# Autodesk Inventor assembly: stratos_v2_mechanics
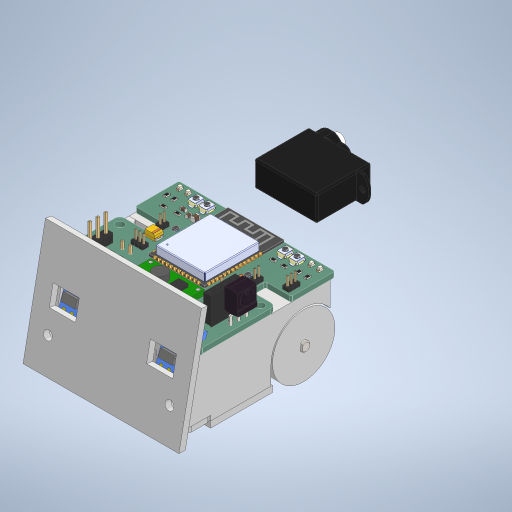
[picture p0: Inventor's stored thumbnail of the model, 512x512]
Saved by Autodesk Inventor 2023.5 (Build 275446000, 446)
## iProperties
Created: 2025-03-17
Part Number: stratos_v2_mechanics
Document SubType Name: Assembly
Designer: kamil
Author: kamil
## Documents named in this file (15)
- E:\PROJECTS_REPOS\Stratos---MicroSumo\mechanics\mechanics V2\stratos_v2_mechanics.iam
- E:\PROJECTS_REPOS\Stratos---MicroSumo\mechanics\Microsumo\mocowanie.ipt
- E:\PROJECTS_REPOS\Stratos---MicroSumo\mechanics\Microsumo\silnik.ipt
- E:\PROJECTS_REPOS\Stratos---MicroSumo\mechanics\mechanics V2\kolo.ipt
- E:\PROJECTS_REPOS\Stratos---MicroSumo\mechanics\mechanics V2\lipo-300.ipt
- E:\PROJECTS_REPOS\Stratos---MicroSumo\mechanics\mechanics V2\MikroSumo\MikroSumo.ipt
- E:\PROJECTS_REPOS\Stratos---MicroSumo\mechanics\mechanics V2\wymiar.ipt
- E:\PROJECTS_REPOS\Stratos---MicroSumo\mechanics\pcb_dolne.ipt
- E:\PROJECTS_REPOS\Stratos---MicroSumo\mechanics\servo_mini_1370hd_cos.ipt
- E:\PROJECTS_REPOS\Stratos---MicroSumo\mechanics\mechanics V2\podstawa_v2.ipt
- E:\PROJECTS_REPOS\Stratos---MicroSumo\mechanics\Microsumo\zebatka_kolo.ipt
- E:\PROJECTS_REPOS\Stratos---MicroSumo\mechanics\Microsumo\zebatka_montaz.ipt
- E:\PROJECTS_REPOS\Stratos---MicroSumo\mechanics\Microsumo\montaz_osi.ipt
- E:\PROJECTS_REPOS\Stratos---MicroSumo\mechanics\Microsumo\nozzyk.ipt
- E:\PROJECTS_REPOS\Stratos---MicroSumo\mechanics\Microsumo\scianka_prawa.ipt
## Components (16 placed, 14 different names)
1. mocowanie:1 — Zestawiające:2, Zestawiające:6, Zestawiające:19, Zestawiające:20
2. silnik:1 — Zestawiające:1, Kątowe:1, Równoległe:1, Zestawiające:2, Równoległe:3, Zestawiające:5
3. silnik:2 — Zestawiające:1, Kątowe:1, Równoległe:1, Równoległe:3, Kątowe:4, Równoległe:9, Zestawiające:14, Zestawiające:17, Zestawiające:18, Kątowe:6
4. kolo:1 — Zestawiające:5, Zestawiające:7
5. kolo:2 — Zestawiające:6, Zestawiające:7, Równoległe:7, Równoległe:8, Zestawiające:12, Zestawiające:13
6. lipo-300:1 — Równoległe:9, Kątowe:5, Zestawiające:17, Równoległe:19, Zestawiające:23, Równoległe:23
7. MikroSumo:1 — Równoległe:7, Kątowe:5, Równoległe:18, Zestawiające:23
8. wymiar:1 — Równoległe:8, Zestawiające:12, Zestawiające:13, Kątowe:4, Równoległe:16, Równoległe:18, Równoległe:19, Równoległe:20
9. pcb_dolne:1 — Zestawiające:25, Równoległe:22, Równoległe:23
10. servo_mini_1370hd_cos:2
11. podstawa_v2:1 — Zestawiające:14, Równoległe:16, Zestawiające:22, Równoległe:21
12. zebatka_kolo:1 — Zestawiające:19, Zestawiające:21
13. zebatka_montaz:1 — Zestawiające:18, Kątowe:6
14. montaz_osi:1 — Zestawiające:20, Zestawiające:21, Zestawiające:22
15. nozzyk:1 — Równoległe:20, Zestawiające:25, Równoległe:22
16. scianka_prawa:1 — Równoległe:21
## Relationships (32: Mate 16, Flush 12, Angle 4)
- Zestawiające:1 [Mate]: silnik:1 ↔ silnik:2
- Kątowe:1 [Angle] (180 deg): silnik:1 ↔ silnik:2
- Równoległe:1 [Flush]: silnik:1 ↔ silnik:2
- Zestawiające:2 [Mate]: mocowanie:1 ↔ silnik:1
- Równoległe:3 [Flush] (1 mm): silnik:1 ↔ silnik:2
- Zestawiające:5 [Mate]: silnik:1 ↔ kolo:1
- Zestawiające:6 [Mate]: mocowanie:1 ↔ kolo:2
- Zestawiające:7 [Mate] (-50 mm): kolo:1 ↔ kolo:2
- Równoległe:7 [Flush]: kolo:2 ↔ MikroSumo:1
- Równoległe:8 [Flush]: kolo:2 ↔ wymiar:1
- Zestawiające:12 [Mate] (-10 mm): kolo:2 ↔ wymiar:1
- Zestawiające:13 [Mate] (-10 mm): kolo:2 ↔ wymiar:1
- Kątowe:4 [Angle] (0 deg): silnik:2 ↔ wymiar:1
- Równoległe:9 [Flush]: silnik:2 ↔ lipo-300:1
- Kątowe:5 [Angle] (180 deg): lipo-300:1 ↔ MikroSumo:1
- Zestawiające:14 [Mate]: silnik:2 ↔ podstawa_v2:1
- Równoległe:16 [Flush]: wymiar:1 ↔ podstawa_v2:1
- Zestawiające:17 [Mate] (1 mm): silnik:2 ↔ lipo-300:1
- Zestawiające:18 [Mate]: silnik:2 ↔ zebatka_montaz:1
- Zestawiające:19 [Mate]: mocowanie:1 ↔ zebatka_kolo:1
- Kątowe:6 [Angle] (180 deg): silnik:2 ↔ zebatka_montaz:1
- Zestawiające:20 [Mate]: mocowanie:1 ↔ montaz_osi:1
- Zestawiające:21 [Mate] (0.2 mm): zebatka_kolo:1 ↔ montaz_osi:1
- Zestawiające:22 [Mate]: podstawa_v2:1 ↔ montaz_osi:1
- Równoległe:18 [Flush]: MikroSumo:1 ↔ wymiar:1
- Równoległe:19 [Flush] (-5.5 mm): lipo-300:1 ↔ wymiar:1
- Zestawiające:23 [Mate] (2 mm): lipo-300:1 ↔ MikroSumo:1
- Równoległe:20 [Flush]: wymiar:1 ↔ nozzyk:1
- Równoległe:21 [Flush]: podstawa_v2:1 ↔ scianka_prawa:1
- Zestawiające:25 [Mate]: pcb_dolne:1 ↔ nozzyk:1
- Równoległe:22 [Flush]: pcb_dolne:1 ↔ nozzyk:1
- Równoległe:23 [Flush]: lipo-300:1 ↔ pcb_dolne:1
